# Autodesk Inventor assembly: Eje delantero _1_
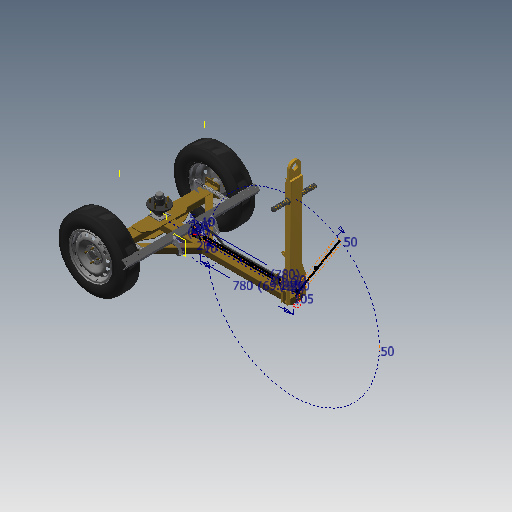
[picture p0: Inventor's stored thumbnail of the model, 512x512]
Saved by Autodesk Inventor 2020 (Build 240168000, 168)
## iProperties
Created: 2020-02-06
Part Number: Eje delantero _1_
Document SubType Name: Assembly
Designer: Juan Carlos Botero
Mass: 142961 g
Surface Area: 67933.4 cm^2
Volume: 18859.4 cm^3
Density: 7.58034 g/cm^3
Author: Juan Carlos Botero
## Documents named in this file (26)
- D:\Drives\OneDrive\Carlos_2\02 TRABAJOS\MULTIPLO\Conveyor\ENSAMBLE\Eje delantero _1_.iam
- D:\Drives\OneDrive\Carlos_2\02 TRABAJOS\MULTIPLO\Conveyor\ENSAMBLE\Seguro de tiro.ipt
- D:\Drives\OneDrive\Carlos_2\02 TRABAJOS\MULTIPLO\Conveyor\ENSAMBLE\Lamina bocin rueda.ipt
- D:\Drives\OneDrive\Carlos_2\02 TRABAJOS\MULTIPLO\Conveyor\ENSAMBLE\Lamina refuerzo eje quinta rueda.ipt
- D:\Drives\OneDrive\Carlos_2\02 TRABAJOS\MULTIPLO\Conveyor\ENSAMBLE\Lamina refuerzo tiro.ipt
- D:\Drives\OneDrive\Carlos_2\02 TRABAJOS\MULTIPLO\Conveyor\ENSAMBLE\Perfil tiro.ipt
- D:\Drives\OneDrive\Carlos_2\02 TRABAJOS\MULTIPLO\Conveyor\ENSAMBLE\Espaciador de nylon.ipt
- D:\Drives\OneDrive\Carlos_2\02 TRABAJOS\MULTIPLO\Conveyor\ENSAMBLE\Arandela de nylon (1).ipt
- D:\Drives\OneDrive\Carlos_2\02 TRABAJOS\MULTIPLO\Conveyor\ENSAMBLE\Refuerzo diagonal tiro (1).ipt
- D:\Drives\OneDrive\Carlos_2\02 TRABAJOS\MULTIPLO\Conveyor\ENSAMBLE\Barra quinta rueda.ipt
- D:\Drives\OneDrive\Carlos_2\02 TRABAJOS\MULTIPLO\Conveyor\ENSAMBLE\Lamina pivote seguro tiro.ipt
- D:\Drives\OneDrive\Carlos_2\02 TRABAJOS\MULTIPLO\Conveyor\ENSAMBLE\Tapa perfiles tiro.ipt
- D:\Drives\OneDrive\Carlos_2\02 TRABAJOS\MULTIPLO\Conveyor\ENSAMBLE\Rin 13_.ipt
- D:\Drives\OneDrive\Carlos_2\02 TRABAJOS\MULTIPLO\Conveyor\ENSAMBLE\70 R13.ipt
- D:\Drives\OneDrive\Carlos_2\02 TRABAJOS\MULTIPLO\Conveyor\ENSAMBLE\Bocin llantas _2_.iam
- D:\Drives\OneDrive\Carlos_2\02 TRABAJOS\MULTIPLO\Conveyor\ENSAMBLE\Bocin eje quinta rueda _1_.iam
- D:\Drives\OneDrive\Carlos_2\02 TRABAJOS\MULTIPLO\Conveyor\ENSAMBLE\Bocin llantas _1_.iam
- D:\Drives\OneDrive\Carlos_2\02 TRABAJOS\MULTIPLO\Conveyor\ENSAMBLE\Soporte freno.ipt
- D:\Drives\OneDrive\Carlos_2\02 TRABAJOS\MULTIPLO\Conveyor\ENSAMBLE\Soporte pivote freno.ipt
- D:\Drives\OneDrive\Carlos_2\02 TRABAJOS\MULTIPLO\Conveyor\ENSAMBLE\Manillar_freno.iam
- D:\Drives\OneDrive\Carlos_2\02 TRABAJOS\MULTIPLO\Conveyor\ENSAMBLE - Copy\Link_bar.ipt
- D:\Drives\OneDrive\Carlos_2\02 TRABAJOS\MULTIPLO\Conveyor\ENSAMBLE - Copy\Tensor_.iam
- D:\Drives\OneDrive\Carlos_2\02 TRABAJOS\MULTIPLO\Conveyor\ENSAMBLE - Copy\Barra freno_W.iam
- D:\Drives\OneDrive\Carlos_2\02 TRABAJOS\MULTIPLO\Conveyor\ENSAMBLE\Eje delantero _1_\Design Accelerator\Bolted Connection3.iam
- D:\Drives\OneDrive\Carlos_2\02 TRABAJOS\MULTIPLO\Conveyor\ENSAMBLE\Eje delantero _1_\Design Accelerator\Bolted Connection4.iam
- D:\Drives\OneDrive\Carlos_2\02 TRABAJOS\MULTIPLO\Conveyor\ENSAMBLE\Eje delantero _1_\Design Accelerator\Bolted Connection5.iam
## Components (37 placed, 23 different names)
1. Seguro de tiro:1
2. Lamina bocin rueda:1 — Symmetry:1, Mate:48
3. Lamina refuerzo eje quinta rueda:1
4. Lamina refuerzo eje quinta rueda:2
5. Perfil tiro:1 — Angle:2
6. Espaciador de nylon:11
7. Lamina refuerzo tiro:3
8. Arandela de nylon (1):1
9. Arandela de nylon (1):2
10. Refuerzo diagonal tiro (1):1
11. Barra quinta rueda:1 — Mate:27, Flush:3
12. Lamina pivote seguro tiro:1
13. Refuerzo diagonal tiro (1):2 — Flush:4
14. Lamina pivote seguro tiro:2
15. Tapa perfiles tiro:2
16. Lamina bocin rueda:2 — Symmetry:1, Mate:47
17. Espaciador de nylon:12
18. Rin 13":3
19. 70 R13:3
20. Lamina refuerzo tiro:6
21. 70 R13:4
22. Rin 13":4
23. Bocin llantas <2>:1 [sub-assembly]
24. Bocin eje quinta rueda <1>:1 [sub-assembly]
25. Bocin llantas <1>:1 [sub-assembly]
26. Soporte freno:1 — Mate:8
27. Soporte pivote freno:1 — Mate:37, Mate:39
28. Soporte pivote freno:2 — Mate:38, Mate:40, Flush:4
29. Manillar_freno:1 [sub-assembly] — Angle:2, Mate:26, Mate:45, Mate:46
30. Link_bar:1 — Mate:26, Rotational:6
31. Tensor_:1 [sub-assembly] — Flush:1, Flush:2, Mate:27, Flush:3, Mate:48
32. Tensor_:2 [sub-assembly] — Flush:1, Flush:2, Mate:47
33. Barra freno_W:1 [sub-assembly] — Rotational:6, Mate:37, Mate:38, Mate:39, Mate:40, Mate:41, Mate:42, Mate:43, Mate:44, Rotational:7
34. Bolted Connection:1 [sub-assembly] — Mate:41, Mate:42
35. Bolted Connection:2 [sub-assembly] — Mate:43, Mate:44
36. Bolted Connection:3 [sub-assembly] — Mate:45, Mate:46
37. Bolted Connection:4 [sub-assembly] — Rotational:7
## Relationships (24: Mate 15, Flush 4, RevoluteJoint 3, Symmetry 1, Angle 1)
- Symmetry:1: Lamina bocin rueda:1 ↔ Lamina bocin rueda:2
- Mate:8: Soporte freno:1
- [RevoluteJoint]: Espaciador de nylon:12 ↔ Manillar_freno:1
- Angle:2 (90 deg): Perfil tiro:1 ↔ Manillar_freno:1
- Mate:26: Manillar_freno:1 ↔ Link_bar:1
- Rotational:6 [RevoluteJoint] (-4 mm): Link_bar:1 ↔ Barra freno_W:1
- Flush:1: Tensor_:1 ↔ Tensor_:2
- Flush:2: Tensor_:1 ↔ Tensor_:2
- Mate:27: Barra quinta rueda:1 ↔ Tensor_:1
- Flush:3: Barra quinta rueda:1 ↔ Tensor_:1
- Mate:37: Soporte pivote freno:1 ↔ Barra freno_W:1
- Mate:38: Soporte pivote freno:2 ↔ Barra freno_W:1
- Mate:39 (3 mm): Soporte pivote freno:1 ↔ Barra freno_W:1
- Mate:40 (3 mm): Soporte pivote freno:2 ↔ Barra freno_W:1
- Mate:41: Barra freno_W:1 ↔ Bolted Connection:1
- Mate:42: Barra freno_W:1 ↔ Bolted Connection:1
- Mate:43: Barra freno_W:1 ↔ Bolted Connection:2
- Mate:44: Barra freno_W:1 ↔ Bolted Connection:2
- Mate:45: Manillar_freno:1 ↔ Bolted Connection:3
- Mate:46: Manillar_freno:1 ↔ Bolted Connection:3
- Flush:4 (25 mm): Refuerzo diagonal tiro (1):2 ↔ Soporte pivote freno:2
- Rotational:7 [RevoluteJoint]: Barra freno_W:1 ↔ Bolted Connection:4
- Mate:47 (60 mm): Lamina bocin rueda:2 ↔ Tensor_:2
- Mate:48 (60 mm): Lamina bocin rueda:1 ↔ Tensor_:1
